# Autodesk Inventor assembly: Cam_assembly
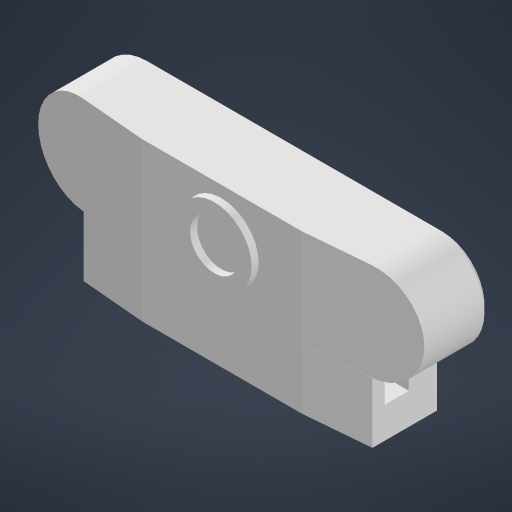
[picture p0: Inventor's stored thumbnail of the model, 512x512]
Saved by Autodesk Inventor 2024 (Build 280153000, 153)
## iProperties
Created: 2025-09-25
Part Number: Cam_assembly
Document SubType Name: Assembly
Designer: kevin
Author: kevin
## Documents named in this file (3)
- C:\Users\kevin\Desktop\SeniorDesign\Head_V3\Cam_assembly.iam
- C:\Users\kevin\Desktop\SeniorDesign\Head_V3\Camera_Clip.ipt
- C:\Users\kevin\Desktop\SeniorDesign\Emeet_Camera.ipt
## Components (2 placed, 2 different names)
1. Camera_Clip:1 — Mate:1, Flush:1, Flush:2
2. Emeet_Camera:1 — Mate:1, Flush:1, Flush:2
## Relationships (3: Flush 2, Mate 1)
- Mate:1: Camera_Clip:1 ↔ Emeet_Camera:1
- Flush:1: Camera_Clip:1 ↔ Emeet_Camera:1
- Flush:2: Camera_Clip:1 ↔ Emeet_Camera:1
